# Autodesk Inventor assembly: (Unsaved)
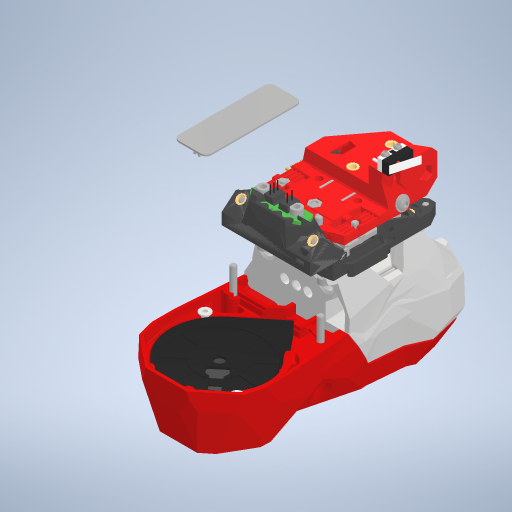
[picture p0: Inventor's stored thumbnail of the model, 512x512]
Saved by Autodesk Inventor 2024 (Build 280153020, 153B)
## iProperties
Created: 2023-06-23
Part Number: (Unsaved)
Document SubType Name: Assembly
Designer: torban
Sending System: Autodesk Translation Framework v12.6.0.85
Preprocessor: ST-DEVELOPER v19.2
Title: Stealthburner_CW2_Assembly.step
## Documents named in this file (8)
- D:\GIT\Voron-Stealthburner\CAD\TORBANMASHUP.iam
- D:\GIT\Voron-Stealthburner\CAD\Stealthburner_CW2_Assembly\Stealthburner_Assembly.iam
- D:\GIT\Voron-Stealthburner\CAD\Stealthburner_CW2_Assembly\ADXL_Assembly - Generic.iam
- D:\GIT\Voron-Stealthburner\CAD\Stealthburner_CW2_Assembly\X_Carriage.iam
- D:\GIT\Voron-Tap\CAD\VORON_Tap_R8\VORON_Tap_R8.iam
- D:\GIT\Voron-Stealthburner\CAD\mosquitto\voron-stealthburner-slice-engineering-mosquito-model_files\high_Mosquito_Voron_TH Rear CW2\high_Mosquito_Voron_TH Rear CW2.ipt
- D:\GIT\Voron-Stealthburner\CAD\mosquitto\voron-stealthburner-slice-engineering-mosquito-model_files\high_Mosquito_Voron_TH_Front\high_Mosquito_Voron_TH_Front.ipt
- D:\GIT\Voron-Stealthburner\CAD\mosquito-hotend-1.snapshot.1\MOSQUITO_HOTEND\MOSQUITO_HOTEND.ipt
## Components (7 placed, 7 different names)
1. Stealthburner_Assembly:1 [sub-assembly] — Mate:13, Mate:14, Mate:15
2. ADXL_Assembly - Generic:1 [sub-assembly]
3. X_Carriage:1 [sub-assembly]
4. VORON_Tap_R8:1 [sub-assembly] — Mate:10, Mate:11, Mate:12
5. high_Mosquito_Voron_TH Rear CW2:1 — Mate:10, Mate:11, Mate:12, Mate:13, Mate:14, Mate:15, Mate:19, Mate:20, Mate:21, Mate:22, Mate:23
6. high_Mosquito_Voron_TH_Front:1 — Mate:19, Mate:20, Mate:21
7. MOSQUITO_HOTEND:1 — Mate:22, Mate:23
## Relationships (11: Mate 11)
- Mate:10: VORON_Tap_R8:1 ↔ high_Mosquito_Voron_TH Rear CW2:1
- Mate:11: VORON_Tap_R8:1 ↔ high_Mosquito_Voron_TH Rear CW2:1
- Mate:12: VORON_Tap_R8:1 ↔ high_Mosquito_Voron_TH Rear CW2:1
- Mate:13: Stealthburner_Assembly:1 ↔ high_Mosquito_Voron_TH Rear CW2:1
- Mate:14: Stealthburner_Assembly:1 ↔ high_Mosquito_Voron_TH Rear CW2:1
- Mate:15: Stealthburner_Assembly:1 ↔ high_Mosquito_Voron_TH Rear CW2:1
- Mate:19: high_Mosquito_Voron_TH Rear CW2:1 ↔ high_Mosquito_Voron_TH_Front:1
- Mate:20: high_Mosquito_Voron_TH Rear CW2:1 ↔ high_Mosquito_Voron_TH_Front:1
- Mate:21: high_Mosquito_Voron_TH Rear CW2:1 ↔ high_Mosquito_Voron_TH_Front:1
- Mate:22: high_Mosquito_Voron_TH Rear CW2:1 ↔ MOSQUITO_HOTEND:1
- Mate:23: high_Mosquito_Voron_TH Rear CW2:1 ↔ MOSQUITO_HOTEND:1
